# Autodesk Inventor assembly: microservoAssembly
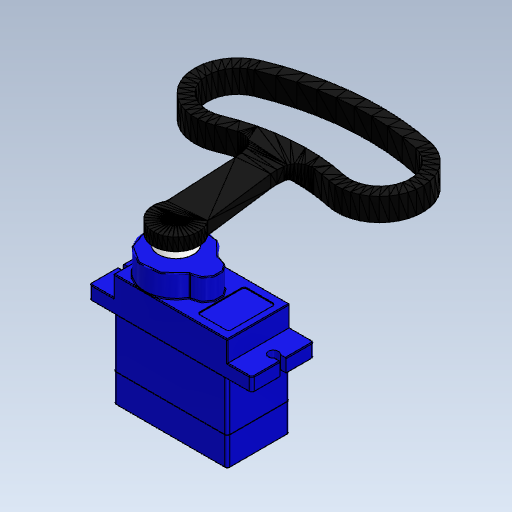
[picture p0: Inventor's stored thumbnail of the model, 512x512]
Saved by Autodesk Inventor 2020.2 (Build 242310000, 310)
## iProperties
Created: 2019-10-25
Part Number: microservoAssembly
Description: STEP AP214
Document SubType Name: Assembly
Designer: Haashim Rehan
Sending System: SolidWorks 2018
Preprocessor: SwSTEP 2.0
Title: microservoAssembly.STEP
Revision Number: ANY
## Documents named in this file (4)
- C:\Users\Dell\Documents\GitHub\Automatic-Light-Switch\CAD\Servo\microservoAssembly.iam
- C:\Users\Dell\Documents\GitHub\Automatic-Light-Switch\CAD\Servo\microservoSG90.ipt
- C:\Users\Dell\Documents\GitHub\Automatic-Light-Switch\CAD\Servo\microservoArm_A2.ipt
- C:\Users\Dell\Documents\GitHub\Automatic-Light-Switch\CAD\Servo\ble_servo_arm.ipt
## Components (3 placed, 3 different names)
1. microservoSG90_1 — Mate:1, Mate:2
2. microservoArm_A2_2 — Mate:1, Mate:2, Mate:3, Mate:4, Angle:1
3. ble_servo_arm:1 — Mate:3, Mate:4, Angle:1
## Relationships (5: Mate 4, Angle 1)
- Mate:1: microservoSG90_1 ↔ microservoArm_A2_2
- Mate:2: microservoSG90_1 ↔ microservoArm_A2_2
- Mate:3: microservoArm_A2_2 ↔ ble_servo_arm:1
- Mate:4: microservoArm_A2_2 ↔ ble_servo_arm:1
- Angle:1 (-2 deg): microservoArm_A2_2 ↔ ble_servo_arm:1
